# Autodesk Inventor assembly: testframe
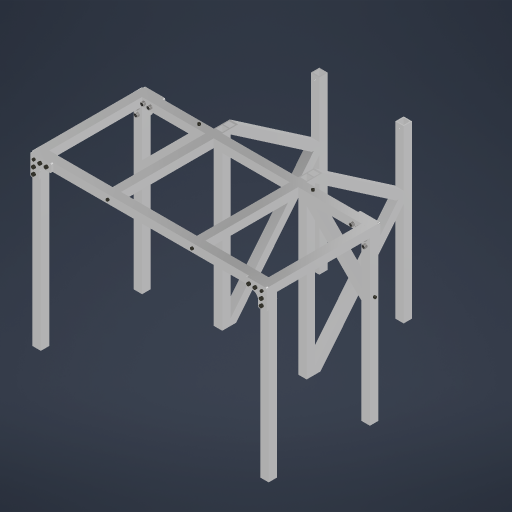
[picture p0: Inventor's stored thumbnail of the model, 512x512]
Saved by Autodesk Inventor 2024.2 (Build 282272000, 272)
## iProperties
Created: 2024-07-23
Part Number: testframe
Document SubType Name: Assembly
Designer: bryan
Mass: 4656.84 g
Surface Area: 9721.76 cm^2
Volume: 1652.17 cm^3
Density: 2.81863 g/cm^3
Author: bryan
## Documents named in this file (24)
- C:\Users\bobsb\OneDrive\Documents\GitHub\1622-2024-Summer-CAD-A-Thon\Structure\STRU_000_StructureAssembly.iam
- C:\Users\bobsb\OneDrive\Documents\GitHub\1622-2024-Summer-CAD-A-Thon\Structure\STRU_001_BilletBlock.ipt
- C:\Users\bobsb\OneDrive\Documents\GitHub\1622-2024-Summer-CAD-A-Thon\Structure\STRU_002_BilletPole_20.56in_Angled.ipt
- C:\Users\bobsb\OneDrive\Documents\GitHub\1622-2024-Summer-CAD-A-Thon\Structure\STRU_003_BilletPole_28in_Angled.ipt
- C:\Users\bobsb\OneDrive\Documents\GitHub\1622-2024-Summer-CAD-A-Thon\Structure\STRU_004_DoubleBillet_90_2.25in.ipt
- C:\Users\bobsb\OneDrive\Documents\GitHub\1622-2024-Summer-CAD-A-Thon\Structure\STRU_007_BilletPole_11in.ipt
- C:\Users\bobsb\OneDrive\Documents\GitHub\1622-2024-Summer-CAD-A-Thon\Structure\STRU_003_BilletPole_28in_Angled_Unique.ipt
- C:\Users\bobsb\OneDrive\Documents\GitHub\1622-2024-Summer-CAD-A-Thon\COTS Library\Fasteners\Bolts\Socket-Head\10-32\COTS_90044A120_Black-Oxide Alloy Steel Socket Head Screw.ipt
- C:\Users\bobsb\OneDrive\Documents\GitHub\1622-2024-Summer-CAD-A-Thon\COTS Library\Fasteners\Bolts\Socket-Head\0.25-20\COTS_90044A123_Black-Oxide Alloy Steel Socket Head Screw.ipt
- C:\Users\bobsb\OneDrive\Documents\GitHub\1622-2024-Summer-CAD-A-Thon\COTS Library\Fasteners\Nuts\COTS_95615A120_Medium-Strength Steel Nylon-Insert Locknut.ipt
- C:\Users\bobsb\OneDrive\Documents\GitHub\1622-2024-Summer-CAD-A-Thon\Structure\STRU_009_FrameBracket_90.ipt
- C:\Users\bobsb\OneDrive\Documents\GitHub\1622-2024-Summer-CAD-A-Thon\Structure\STRU_006_BilletPole_SwerveOffset.ipt
- C:\Users\bobsb\OneDrive\Documents\GitHub\1622-2024-Summer-CAD-A-Thon\Structure\STRU_010_BilletCrossbar_Angled.ipt
- C:\Users\bobsb\OneDrive\Documents\GitHub\1622-2024-Summer-CAD-A-Thon\Structure\STRU_011_BilletWedge.ipt
- C:\Users\bobsb\OneDrive\Documents\GitHub\1622-2024-Summer-CAD-A-Thon\COTS Library\Fasteners\Bolts\Socket-Head\10-32\COTS_90044A119_Black-Oxide Alloy Steel Socket Head Screw.ipt
- C:\Users\bobsb\OneDrive\Documents\GitHub\1622-2024-Summer-CAD-A-Thon\Structure\STRU_012_BilletPoleMiddle.ipt
- C:\Users\bobsb\OneDrive\Documents\GitHub\1622-2024-Summer-CAD-A-Thon\Structure\STRU_013_BilletCrossbar2_Angled.ipt
- C:\Users\bobsb\OneDrive\Documents\GitHub\1622-2024-Summer-CAD-A-Thon\Structure\STRU_014_BilletCrossbar3_Angled.ipt
- C:\Users\bobsb\OneDrive\Documents\GitHub\1622-2024-Summer-CAD-A-Thon\Structure\STRU_000_StructureAssembly\AIP\FEA\err5tqx4w.fins
- C:\Users\bobsb\OneDrive\Documents\GitHub\1622-2024-Summer-CAD-A-Thon\Structure\STRU_000_StructureAssembly\AIP\FEA\err5tqx4w.fsat
- C:\Users\bobsb\OneDrive\Documents\GitHub\1622-2024-Summer-CAD-A-Thon\Structure\STRU_000_StructureAssembly\AIP\FEA\err5tqx4w.ftes
- C:\Users\bobsb\OneDrive\Documents\GitHub\1622-2024-Summer-CAD-A-Thon\Structure\STRU_000_StructureAssembly\AIP\FEA\err5tqx5s.fwiz
- C:\Users\bobsb\OneDrive\Documents\GitHub\1622-2024-Summer-CAD-A-Thon\Structure\STRU_000_StructureAssembly\AIP\FEA\err5tqxb4.fmsh
- C:\Users\bobsb\OneDrive\Documents\GitHub\1622-2024-Summer-CAD-A-Thon\Structure\STRU_000_StructureAssembly\AIP\FEA\err5tqxb5.fres
## Components (90 placed, 17 different names)
1. STRU_001_BilletBlock:2 — Mate:16, Mate:17, Flush:2
2. STRU_002_BilletPole_20.56in_Angled:1 — Mate:1, Mate:4, Mate:5, Mate:41, Mate:53, Mate:54, Flush:10, Mate:91, Mate:92, Mate:127, Mate:147, Mate:148, Mate:199, Mate:209, Mate:211, Mate:212, Mate:213
3. STRU_004_DoubleBillet_90_2.25in:1 — Mate:1, Mate:4, Mate:5, Mate:34, Mate:56, Mate:58, Mate:125, Mate:126
4. STRU_002_BilletPole_20.56in_Angled:2 — Mate:13, Mate:14, Mate:15, Mate:16, Mate:17, Flush:2, Mate:40, Mate:85, Mate:86, Mate:123, Mate:124, Mate:145, Mate:146, Mate:197, Mate:200, Mate:201, Mate:218, Mate:219
5. STRU_004_DoubleBillet_90_2.25in:2 — Mate:13, Mate:14, Mate:15, Mate:36, Mate:57, Mate:100, Mate:121, Mate:122
6. STRU_001_BilletBlock:3 — Mate:185, Mate:186, Flush:26
7. STRU_001_BilletBlock:4 — Mate:180, Mate:181, Flush:25
8. STRU_003_BilletPole_28in_Angled:2 — Mate:47, Flush:8, Flush:9, Mate:55, Mate:74, Mate:79, Mate:80, Mate:87, Mate:88, Mate:97, Mate:118, Mate:130, Mate:140, Mate:153, Mate:154, Mate:155, Mate:156, Mate:157, Mate:158, Mate:161, Mate:163, Mate:168, Mate:173, Flush:24, Mate:176, Mate:178, Mate:182
9. STRU_004_DoubleBillet_90_2.25in:3 — Mate:35, Mate:128, Mate:129, Mate:184
10. STRU_004_DoubleBillet_90_2.25in:4 — Mate:37, Mate:119, Mate:120, Mate:179
11. STRU_001_BilletBlock:5 — Mate:34, Mate:41, Mate:50, Mate:51
12. STRU_001_BilletBlock:6 — Mate:35, Mate:48, Mate:49
13. STRU_001_BilletBlock:7 — Mate:37, Mate:45, Mate:46
14. STRU_001_BilletBlock:8 — Mate:36, Mate:40, Mate:42, Mate:43
15. STRU_007_BilletPole_11in:1 — Mate:48, Mate:49, Flush:9, Mate:50, Mate:51, Mate:55, Mate:59
16. STRU_007_BilletPole_11in:2 — Mate:42, Mate:43, Mate:45, Mate:46, Mate:47, Flush:8, Mate:124
17. STRU_001_BilletBlock:9 — Mate:53, Mate:54, Flush:10
18. STRU_003_BilletPole_28in_Angled_Unique:1 — Mate:56, Mate:57, Mate:58, Mate:59, Mate:83, Mate:84, Mate:93, Mate:94, Mate:98, Mate:149, Mate:150, Mate:151, Mate:152, Mate:159, Mate:160, Mate:164, Mate:165, Mate:196, Mate:198, Flush:27, Mate:203, Mate:205, Mate:206, Mate:208, Mate:214, Mate:215, Mate:216, Mate:217, Mate:220, Flush:28, Mate:221, Mate:222, Flush:29, Mate:223, Flush:35, Mate:232
19. STRU_001_BilletBlock:10 — Mate:74, Mate:157, Mate:172
20. COTS_90044A120_Black-Oxide Alloy Steel Socket Head Screw:1 — Mate:142, Mate:193
21. COTS_90044A123_Black-Oxide Alloy Steel Socket Head Screw:2 — Mate:80, Mate:102, Mate:141, Flush:21
22. COTS_90044A123_Black-Oxide Alloy Steel Socket Head Screw:3 — Mate:103, Flush:22, Flush:23, Mate:191
23. COTS_90044A123_Black-Oxide Alloy Steel Socket Head Screw:4 — Mate:79, Mate:101, Flush:21, Flush:22
24. COTS_90044A123_Black-Oxide Alloy Steel Socket Head Screw:5 — Mate:104, Flush:23, Mate:192
25. COTS_90044A123_Black-Oxide Alloy Steel Socket Head Screw:6 — Mate:84, Mate:108, Flush:12
26. COTS_90044A123_Black-Oxide Alloy Steel Socket Head Screw:7 — Mate:85, Mate:106, Mate:134, Flush:12, Flush:13, Flush:14
27. COTS_90044A123_Black-Oxide Alloy Steel Socket Head Screw:8 — Mate:83, Mate:107, Flush:13
28. COTS_90044A123_Black-Oxide Alloy Steel Socket Head Screw:9 — Mate:86, Mate:105, Flush:14
29. COTS_90044A123_Black-Oxide Alloy Steel Socket Head Screw:10 — Mate:112, Flush:18, Mate:188
30. COTS_90044A123_Black-Oxide Alloy Steel Socket Head Screw:11 — Mate:111, Mate:139, Flush:18, Flush:19, Flush:20, Mate:187
31. COTS_90044A123_Black-Oxide Alloy Steel Socket Head Screw:12 — Mate:88, Mate:110, Flush:20
32. COTS_90044A123_Black-Oxide Alloy Steel Socket Head Screw:13 — Mate:87, Mate:109, Flush:19
33. COTS_90044A123_Black-Oxide Alloy Steel Socket Head Screw:14 — Mate:93, Mate:115, Flush:16
34. COTS_90044A123_Black-Oxide Alloy Steel Socket Head Screw:15 — Mate:92, Mate:114, Flush:17
35. COTS_90044A123_Black-Oxide Alloy Steel Socket Head Screw:16 — Mate:91, Mate:113, Mate:136, Flush:15, Flush:17
36. COTS_90044A123_Black-Oxide Alloy Steel Socket Head Screw:17 — Mate:94, Mate:116, Flush:15, Flush:16
37. COTS_90044A120_Black-Oxide Alloy Steel Socket Head Screw:3 — Mate:140, Mate:158
38. COTS_90044A120_Black-Oxide Alloy Steel Socket Head Screw:5 — Mate:97, Mate:138
39. COTS_90044A120_Black-Oxide Alloy Steel Socket Head Screw:6 — Mate:100, Mate:135
40. COTS_90044A120_Black-Oxide Alloy Steel Socket Head Screw:7 — Mate:98, Mate:137
41. COTS_95615A120_Medium-Strength Steel Nylon-Insert Locknut:1 — Mate:102, Mate:154
42. COTS_95615A120_Medium-Strength Steel Nylon-Insert Locknut:2 — Mate:101, Mate:153
43. COTS_95615A120_Medium-Strength Steel Nylon-Insert Locknut:3 — Mate:103, Mate:194
44. COTS_95615A120_Medium-Strength Steel Nylon-Insert Locknut:4 — Mate:104, Mate:195
45. COTS_95615A120_Medium-Strength Steel Nylon-Insert Locknut:5 — Mate:107, Mate:152
46. COTS_95615A120_Medium-Strength Steel Nylon-Insert Locknut:6 — Mate:108, Mate:151
47. COTS_95615A120_Medium-Strength Steel Nylon-Insert Locknut:7 — Mate:105, Mate:145
48. COTS_95615A120_Medium-Strength Steel Nylon-Insert Locknut:8 — Mate:106, Mate:146
49. COTS_95615A120_Medium-Strength Steel Nylon-Insert Locknut:9 — Mate:109, Mate:155
50. COTS_95615A120_Medium-Strength Steel Nylon-Insert Locknut:10 — Mate:110, Mate:156
51. COTS_95615A120_Medium-Strength Steel Nylon-Insert Locknut:11 — Mate:111, Mate:189
52. COTS_95615A120_Medium-Strength Steel Nylon-Insert Locknut:12 — Mate:112, Mate:190
53. COTS_95615A120_Medium-Strength Steel Nylon-Insert Locknut:13 — Mate:114, Mate:147
54. COTS_95615A120_Medium-Strength Steel Nylon-Insert Locknut:14 — Mate:113, Mate:148
55. COTS_95615A120_Medium-Strength Steel Nylon-Insert Locknut:15 — Mate:115, Mate:149
56. COTS_95615A120_Medium-Strength Steel Nylon-Insert Locknut:16 — Mate:116, Mate:150
57. STRU_009_FrameBracket_90:1 — Mate:118, Mate:119, Mate:120, Mate:141, Mate:142, Mate:177, Mate:191, Mate:192, Mate:193
58. STRU_009_FrameBracket_90:2 — Mate:125, Mate:126, Mate:127, Mate:136, Mate:137
59. STRU_009_FrameBracket_90:3 — Mate:121, Mate:122, Mate:123, Mate:134, Mate:135
60. STRU_009_FrameBracket_90:4 — Mate:128, Mate:129, Mate:130, Mate:138, Mate:139, Mate:183, Mate:187, Mate:188
61. STRU_001_BilletBlock:11 — Mate:159, Mate:165, Mate:171
62. STRU_001_BilletBlock:12 — Mate:160, Mate:164, Mate:174
63. STRU_001_BilletBlock:13 — Mate:161, Mate:162, Mate:163, Mate:175
64. COTS_90044A120_Black-Oxide Alloy Steel Socket Head Screw:10 — Mate:162, Mate:168
65. STRU_007_BilletPole_11in:3 — Mate:171, Mate:172, Mate:173, Flush:27
66. STRU_007_BilletPole_11in:4 — Mate:174, Mate:175, Flush:24, Mate:176
67. STRU_006_BilletPole_SwerveOffset:1 — Mate:177, Mate:178, Mate:179, Mate:180, Mate:181, Flush:25, Mate:194, Mate:195
68. STRU_006_BilletPole_SwerveOffset:2 — Mate:182, Mate:183, Mate:184, Mate:185, Mate:186, Flush:26, Mate:189, Mate:190
69. STRU_010_BilletCrossbar_Angled:1 — Mate:196, Mate:197, Mate:202, Mate:204
70. STRU_010_BilletCrossbar_Angled:2 — Mate:198, Mate:199, Mate:207, Mate:210
71. STRU_011_BilletWedge:1 — Mate:200, Mate:201, Mate:202
72. STRU_011_BilletWedge:3 — Mate:203, Mate:204, Mate:205
73. STRU_011_BilletWedge:4 — Mate:206, Mate:207, Mate:208
74. STRU_011_BilletWedge:5 — Mate:209, Mate:210, Mate:211
75. COTS_90044A119_Black-Oxide Alloy Steel Socket Head Screw:1 — Mate:212, Mate:213
76. COTS_90044A119_Black-Oxide Alloy Steel Socket Head Screw:2 — Mate:214, Mate:215
77. COTS_90044A119_Black-Oxide Alloy Steel Socket Head Screw:3 — Mate:216, Mate:217
78. COTS_90044A119_Black-Oxide Alloy Steel Socket Head Screw:4 — Mate:218, Mate:219
79. STRU_012_BilletPoleMiddle:1 — Mate:220, Flush:28, Mate:221, Mate:228, Mate:229, Flush:30, Flush:34, Flush:43
80. STRU_012_BilletPoleMiddle:2 — Mate:222, Flush:29, Mate:223, Mate:230, Mate:231, Flush:31, Flush:32, Flush:39, Mate:233, Mate:234
81. STRU_001_BilletBlock:14 — Mate:228, Mate:229, Flush:30
82. STRU_001_BilletBlock:15 — Mate:230, Mate:231, Flush:31
83. STRU_012_BilletPoleMiddle:3 — Flush:33, Flush:34, Flush:36, Flush:37, Mate:239, Flush:42, Mate:243, Flush:45, Mate:244, Mate:245, Flush:46
84. STRU_012_BilletPoleMiddle:4 — Flush:32, Flush:33, Flush:35, Flush:36, Mate:232, Flush:37, Mate:241, Flush:44, Mate:246, Mate:247, Flush:47
85. STRU_013_BilletCrossbar2_Angled:1 — Flush:39, Mate:233, Mate:234, Mate:240
86. STRU_013_BilletCrossbar2_Angled:3 — Mate:239, Flush:42, Flush:43, Mate:242
87. STRU_014_BilletCrossbar3_Angled:1 — Mate:240, Mate:241, Flush:44
88. STRU_014_BilletCrossbar3_Angled:2 — Mate:242, Mate:243, Flush:45
89. STRU_001_BilletBlock:16 — Mate:244, Mate:245, Flush:46
90. STRU_001_BilletBlock:17 — Mate:246, Mate:247, Flush:47
## Relationships (218: Mate 181, Flush 37)
- Mate:1: STRU_002_BilletPole_20.56in_Angled:1 ↔ STRU_004_DoubleBillet_90_2.25in:1
- Mate:4: STRU_002_BilletPole_20.56in_Angled:1 ↔ STRU_004_DoubleBillet_90_2.25in:1
- Mate:5: STRU_002_BilletPole_20.56in_Angled:1 ↔ STRU_004_DoubleBillet_90_2.25in:1
- Mate:13: STRU_002_BilletPole_20.56in_Angled:2 ↔ STRU_004_DoubleBillet_90_2.25in:2
- Mate:14: STRU_002_BilletPole_20.56in_Angled:2 ↔ STRU_004_DoubleBillet_90_2.25in:2
- Mate:15: STRU_002_BilletPole_20.56in_Angled:2 ↔ STRU_004_DoubleBillet_90_2.25in:2
- Mate:16: STRU_001_BilletBlock:2 ↔ STRU_002_BilletPole_20.56in_Angled:2
- Mate:17: STRU_001_BilletBlock:2 ↔ STRU_002_BilletPole_20.56in_Angled:2
- Flush:2: STRU_001_BilletBlock:2 ↔ STRU_002_BilletPole_20.56in_Angled:2
- [Mate]: STRU_003_BilletPole_28in_Angled:2 ↔ STRU_004_DoubleBillet_90_2.25in:3
- [Mate]: STRU_003_BilletPole_28in_Angled:2 ↔ STRU_004_DoubleBillet_90_2.25in:3
- [Mate]: STRU_003_BilletPole_28in_Angled:2 ↔ STRU_004_DoubleBillet_90_2.25in:3
- [Mate]: STRU_003_BilletPole_28in_Angled:2 ↔ STRU_004_DoubleBillet_90_2.25in:4
- [Mate]: STRU_003_BilletPole_28in_Angled:2 ↔ STRU_004_DoubleBillet_90_2.25in:4
- [Mate]: STRU_003_BilletPole_28in_Angled:2 ↔ STRU_004_DoubleBillet_90_2.25in:4
- Mate:34: STRU_004_DoubleBillet_90_2.25in:1 ↔ STRU_001_BilletBlock:5
- Mate:35: STRU_004_DoubleBillet_90_2.25in:3 ↔ STRU_001_BilletBlock:6
- Mate:36: STRU_004_DoubleBillet_90_2.25in:2 ↔ STRU_001_BilletBlock:8
- Mate:37: STRU_004_DoubleBillet_90_2.25in:4 ↔ STRU_001_BilletBlock:7
- Mate:40: STRU_002_BilletPole_20.56in_Angled:2 ↔ STRU_001_BilletBlock:8
- Mate:41: STRU_002_BilletPole_20.56in_Angled:1 ↔ STRU_001_BilletBlock:5
- Mate:42: STRU_001_BilletBlock:8 ↔ STRU_007_BilletPole_11in:2
- Mate:43: STRU_001_BilletBlock:8 ↔ STRU_007_BilletPole_11in:2
- Mate:45: STRU_001_BilletBlock:7 ↔ STRU_007_BilletPole_11in:2
- Mate:46: STRU_001_BilletBlock:7 ↔ STRU_007_BilletPole_11in:2
- Mate:47: STRU_003_BilletPole_28in_Angled:2 ↔ STRU_007_BilletPole_11in:2
- Flush:8: STRU_003_BilletPole_28in_Angled:2 ↔ STRU_007_BilletPole_11in:2
- Mate:48: STRU_001_BilletBlock:6 ↔ STRU_007_BilletPole_11in:1
- Mate:49: STRU_001_BilletBlock:6 ↔ STRU_007_BilletPole_11in:1
- Flush:9: STRU_003_BilletPole_28in_Angled:2 ↔ STRU_007_BilletPole_11in:1
- Mate:50: STRU_001_BilletBlock:5 ↔ STRU_007_BilletPole_11in:1
- Mate:51: STRU_001_BilletBlock:5 ↔ STRU_007_BilletPole_11in:1
- Mate:53: STRU_002_BilletPole_20.56in_Angled:1 ↔ STRU_001_BilletBlock:9
- Mate:54: STRU_002_BilletPole_20.56in_Angled:1 ↔ STRU_001_BilletBlock:9
- Flush:10: STRU_002_BilletPole_20.56in_Angled:1 ↔ STRU_001_BilletBlock:9
- Mate:55: STRU_003_BilletPole_28in_Angled:2 ↔ STRU_007_BilletPole_11in:1
- Mate:56: STRU_004_DoubleBillet_90_2.25in:1 ↔ STRU_003_BilletPole_28in_Angled_Unique:1
- Mate:57: STRU_004_DoubleBillet_90_2.25in:2 ↔ STRU_003_BilletPole_28in_Angled_Unique:1
- Mate:58: STRU_004_DoubleBillet_90_2.25in:1 ↔ STRU_003_BilletPole_28in_Angled_Unique:1
- Mate:59: STRU_007_BilletPole_11in:1 ↔ STRU_003_BilletPole_28in_Angled_Unique:1
- Mate:74: STRU_003_BilletPole_28in_Angled:2 ↔ STRU_001_BilletBlock:10
- Mate:79: STRU_003_BilletPole_28in_Angled:2 ↔ COTS_90044A123_Black-Oxide Alloy Steel Socket Head Screw:4
- Mate:80: STRU_003_BilletPole_28in_Angled:2 ↔ COTS_90044A123_Black-Oxide Alloy Steel Socket Head Screw:2
- Mate:83: STRU_003_BilletPole_28in_Angled_Unique:1 ↔ COTS_90044A123_Black-Oxide Alloy Steel Socket Head Screw:8
- Mate:84: STRU_003_BilletPole_28in_Angled_Unique:1 ↔ COTS_90044A123_Black-Oxide Alloy Steel Socket Head Screw:6
- Mate:85: STRU_002_BilletPole_20.56in_Angled:2 ↔ COTS_90044A123_Black-Oxide Alloy Steel Socket Head Screw:7
- Mate:86: STRU_002_BilletPole_20.56in_Angled:2 ↔ COTS_90044A123_Black-Oxide Alloy Steel Socket Head Screw:9
- Mate:87: STRU_003_BilletPole_28in_Angled:2 ↔ COTS_90044A123_Black-Oxide Alloy Steel Socket Head Screw:13
- Mate:88: STRU_003_BilletPole_28in_Angled:2 ↔ COTS_90044A123_Black-Oxide Alloy Steel Socket Head Screw:12
- Mate:91: STRU_002_BilletPole_20.56in_Angled:1 ↔ COTS_90044A123_Black-Oxide Alloy Steel Socket Head Screw:16
- Mate:92: STRU_002_BilletPole_20.56in_Angled:1 ↔ COTS_90044A123_Black-Oxide Alloy Steel Socket Head Screw:15
- Mate:93: STRU_003_BilletPole_28in_Angled_Unique:1 ↔ COTS_90044A123_Black-Oxide Alloy Steel Socket Head Screw:14
- Mate:94: STRU_003_BilletPole_28in_Angled_Unique:1 ↔ COTS_90044A123_Black-Oxide Alloy Steel Socket Head Screw:17
- Mate:97: STRU_003_BilletPole_28in_Angled:2 ↔ COTS_90044A120_Black-Oxide Alloy Steel Socket Head Screw:5
- Mate:98: STRU_003_BilletPole_28in_Angled_Unique:1 ↔ COTS_90044A120_Black-Oxide Alloy Steel Socket Head Screw:7
- Mate:100: STRU_004_DoubleBillet_90_2.25in:2 ↔ COTS_90044A120_Black-Oxide Alloy Steel Socket Head Screw:6
- Mate:101: COTS_90044A123_Black-Oxide Alloy Steel Socket Head Screw:4 ↔ COTS_95615A120_Medium-Strength Steel Nylon-Insert Locknut:2
- Mate:102: COTS_90044A123_Black-Oxide Alloy Steel Socket Head Screw:2 ↔ COTS_95615A120_Medium-Strength Steel Nylon-Insert Locknut:1
- Mate:103: COTS_90044A123_Black-Oxide Alloy Steel Socket Head Screw:3 ↔ COTS_95615A120_Medium-Strength Steel Nylon-Insert Locknut:3
- Mate:104: COTS_90044A123_Black-Oxide Alloy Steel Socket Head Screw:5 ↔ COTS_95615A120_Medium-Strength Steel Nylon-Insert Locknut:4
- Mate:105: COTS_90044A123_Black-Oxide Alloy Steel Socket Head Screw:9 ↔ COTS_95615A120_Medium-Strength Steel Nylon-Insert Locknut:7
- Mate:106: COTS_90044A123_Black-Oxide Alloy Steel Socket Head Screw:7 ↔ COTS_95615A120_Medium-Strength Steel Nylon-Insert Locknut:8
- Mate:107: COTS_90044A123_Black-Oxide Alloy Steel Socket Head Screw:8 ↔ COTS_95615A120_Medium-Strength Steel Nylon-Insert Locknut:5
- Mate:108: COTS_90044A123_Black-Oxide Alloy Steel Socket Head Screw:6 ↔ COTS_95615A120_Medium-Strength Steel Nylon-Insert Locknut:6
- Mate:109: COTS_90044A123_Black-Oxide Alloy Steel Socket Head Screw:13 ↔ COTS_95615A120_Medium-Strength Steel Nylon-Insert Locknut:9
- Mate:110: COTS_90044A123_Black-Oxide Alloy Steel Socket Head Screw:12 ↔ COTS_95615A120_Medium-Strength Steel Nylon-Insert Locknut:10
- Mate:111: COTS_90044A123_Black-Oxide Alloy Steel Socket Head Screw:11 ↔ COTS_95615A120_Medium-Strength Steel Nylon-Insert Locknut:11
- Mate:112: COTS_90044A123_Black-Oxide Alloy Steel Socket Head Screw:10 ↔ COTS_95615A120_Medium-Strength Steel Nylon-Insert Locknut:12
- Mate:113: COTS_90044A123_Black-Oxide Alloy Steel Socket Head Screw:16 ↔ COTS_95615A120_Medium-Strength Steel Nylon-Insert Locknut:14
- Mate:114: COTS_90044A123_Black-Oxide Alloy Steel Socket Head Screw:15 ↔ COTS_95615A120_Medium-Strength Steel Nylon-Insert Locknut:13
- Mate:115: COTS_90044A123_Black-Oxide Alloy Steel Socket Head Screw:14 ↔ COTS_95615A120_Medium-Strength Steel Nylon-Insert Locknut:15
- Mate:116: COTS_90044A123_Black-Oxide Alloy Steel Socket Head Screw:17 ↔ COTS_95615A120_Medium-Strength Steel Nylon-Insert Locknut:16
- Mate:118: STRU_003_BilletPole_28in_Angled:2 ↔ STRU_009_FrameBracket_90:1
- Mate:119: STRU_004_DoubleBillet_90_2.25in:4 ↔ STRU_009_FrameBracket_90:1
- Mate:120: STRU_004_DoubleBillet_90_2.25in:4 ↔ STRU_009_FrameBracket_90:1
- Mate:121: STRU_004_DoubleBillet_90_2.25in:2 ↔ STRU_009_FrameBracket_90:3
- Mate:122: STRU_004_DoubleBillet_90_2.25in:2 ↔ STRU_009_FrameBracket_90:3
- Mate:123: STRU_002_BilletPole_20.56in_Angled:2 ↔ STRU_009_FrameBracket_90:3
- Mate:124: STRU_002_BilletPole_20.56in_Angled:2 ↔ STRU_007_BilletPole_11in:2
- Mate:125: STRU_004_DoubleBillet_90_2.25in:1 ↔ STRU_009_FrameBracket_90:2
- Mate:126: STRU_004_DoubleBillet_90_2.25in:1 ↔ STRU_009_FrameBracket_90:2
- Mate:127: STRU_002_BilletPole_20.56in_Angled:1 ↔ STRU_009_FrameBracket_90:2
- Mate:128: STRU_004_DoubleBillet_90_2.25in:3 ↔ STRU_009_FrameBracket_90:4
- Mate:129: STRU_004_DoubleBillet_90_2.25in:3 ↔ STRU_009_FrameBracket_90:4
- Mate:130: STRU_003_BilletPole_28in_Angled:2 ↔ STRU_009_FrameBracket_90:4
- Mate:134: COTS_90044A123_Black-Oxide Alloy Steel Socket Head Screw:7 ↔ STRU_009_FrameBracket_90:3
- Flush:12: COTS_90044A123_Black-Oxide Alloy Steel Socket Head Screw:6 ↔ COTS_90044A123_Black-Oxide Alloy Steel Socket Head Screw:7
- Mate:135: COTS_90044A120_Black-Oxide Alloy Steel Socket Head Screw:6 ↔ STRU_009_FrameBracket_90:3
- Flush:13: COTS_90044A123_Black-Oxide Alloy Steel Socket Head Screw:7 ↔ COTS_90044A123_Black-Oxide Alloy Steel Socket Head Screw:8
- Flush:14: COTS_90044A123_Black-Oxide Alloy Steel Socket Head Screw:7 ↔ COTS_90044A123_Black-Oxide Alloy Steel Socket Head Screw:9
- Mate:136: COTS_90044A123_Black-Oxide Alloy Steel Socket Head Screw:16 ↔ STRU_009_FrameBracket_90:2
- Mate:137: COTS_90044A120_Black-Oxide Alloy Steel Socket Head Screw:7 ↔ STRU_009_FrameBracket_90:2
- Flush:15: COTS_90044A123_Black-Oxide Alloy Steel Socket Head Screw:16 ↔ COTS_90044A123_Black-Oxide Alloy Steel Socket Head Screw:17
- Flush:16: COTS_90044A123_Black-Oxide Alloy Steel Socket Head Screw:14 ↔ COTS_90044A123_Black-Oxide Alloy Steel Socket Head Screw:17
- Flush:17: COTS_90044A123_Black-Oxide Alloy Steel Socket Head Screw:15 ↔ COTS_90044A123_Black-Oxide Alloy Steel Socket Head Screw:16
- Mate:138: COTS_90044A120_Black-Oxide Alloy Steel Socket Head Screw:5 ↔ STRU_009_FrameBracket_90:4
- Mate:139: COTS_90044A123_Black-Oxide Alloy Steel Socket Head Screw:11 ↔ STRU_009_FrameBracket_90:4
- Flush:18: COTS_90044A123_Black-Oxide Alloy Steel Socket Head Screw:10 ↔ COTS_90044A123_Black-Oxide Alloy Steel Socket Head Screw:11
- Flush:19: COTS_90044A123_Black-Oxide Alloy Steel Socket Head Screw:11 ↔ COTS_90044A123_Black-Oxide Alloy Steel Socket Head Screw:13
- Flush:20: COTS_90044A123_Black-Oxide Alloy Steel Socket Head Screw:11 ↔ COTS_90044A123_Black-Oxide Alloy Steel Socket Head Screw:12
- Mate:140: STRU_003_BilletPole_28in_Angled:2 ↔ COTS_90044A120_Black-Oxide Alloy Steel Socket Head Screw:3
- Mate:141: COTS_90044A123_Black-Oxide Alloy Steel Socket Head Screw:2 ↔ STRU_009_FrameBracket_90:1
- Mate:142: COTS_90044A120_Black-Oxide Alloy Steel Socket Head Screw:1 ↔ STRU_009_FrameBracket_90:1
- Flush:21: COTS_90044A123_Black-Oxide Alloy Steel Socket Head Screw:2 ↔ COTS_90044A123_Black-Oxide Alloy Steel Socket Head Screw:4
- Flush:22: COTS_90044A123_Black-Oxide Alloy Steel Socket Head Screw:3 ↔ COTS_90044A123_Black-Oxide Alloy Steel Socket Head Screw:4
- Flush:23: COTS_90044A123_Black-Oxide Alloy Steel Socket Head Screw:3 ↔ COTS_90044A123_Black-Oxide Alloy Steel Socket Head Screw:5
- Mate:145: STRU_002_BilletPole_20.56in_Angled:2 ↔ COTS_95615A120_Medium-Strength Steel Nylon-Insert Locknut:7
- Mate:146: STRU_002_BilletPole_20.56in_Angled:2 ↔ COTS_95615A120_Medium-Strength Steel Nylon-Insert Locknut:8
- Mate:147: STRU_002_BilletPole_20.56in_Angled:1 ↔ COTS_95615A120_Medium-Strength Steel Nylon-Insert Locknut:13
- Mate:148: STRU_002_BilletPole_20.56in_Angled:1 ↔ COTS_95615A120_Medium-Strength Steel Nylon-Insert Locknut:14
- Mate:149: STRU_003_BilletPole_28in_Angled_Unique:1 ↔ COTS_95615A120_Medium-Strength Steel Nylon-Insert Locknut:15
- Mate:150: STRU_003_BilletPole_28in_Angled_Unique:1 ↔ COTS_95615A120_Medium-Strength Steel Nylon-Insert Locknut:16
- Mate:151: STRU_003_BilletPole_28in_Angled_Unique:1 ↔ COTS_95615A120_Medium-Strength Steel Nylon-Insert Locknut:6
- Mate:152: STRU_003_BilletPole_28in_Angled_Unique:1 ↔ COTS_95615A120_Medium-Strength Steel Nylon-Insert Locknut:5
- Mate:153: STRU_003_BilletPole_28in_Angled:2 ↔ COTS_95615A120_Medium-Strength Steel Nylon-Insert Locknut:2
- Mate:154: STRU_003_BilletPole_28in_Angled:2 ↔ COTS_95615A120_Medium-Strength Steel Nylon-Insert Locknut:1
- Mate:155: STRU_003_BilletPole_28in_Angled:2 ↔ COTS_95615A120_Medium-Strength Steel Nylon-Insert Locknut:9
- Mate:156: STRU_003_BilletPole_28in_Angled:2 ↔ COTS_95615A120_Medium-Strength Steel Nylon-Insert Locknut:10
- Mate:157: STRU_003_BilletPole_28in_Angled:2 ↔ STRU_001_BilletBlock:10
- Mate:158: STRU_003_BilletPole_28in_Angled:2 ↔ COTS_90044A120_Black-Oxide Alloy Steel Socket Head Screw:3
- Mate:159: STRU_003_BilletPole_28in_Angled_Unique:1 ↔ STRU_001_BilletBlock:11
- Mate:160: STRU_003_BilletPole_28in_Angled_Unique:1 ↔ STRU_001_BilletBlock:12
- Mate:161: STRU_003_BilletPole_28in_Angled:2 ↔ STRU_001_BilletBlock:13
- Mate:162: STRU_001_BilletBlock:13 ↔ COTS_90044A120_Black-Oxide Alloy Steel Socket Head Screw:10
- Mate:163: STRU_003_BilletPole_28in_Angled:2 ↔ STRU_001_BilletBlock:13
- Mate:164: STRU_003_BilletPole_28in_Angled_Unique:1 ↔ STRU_001_BilletBlock:12
- Mate:165: STRU_003_BilletPole_28in_Angled_Unique:1 ↔ STRU_001_BilletBlock:11
- Mate:168: STRU_003_BilletPole_28in_Angled:2 ↔ COTS_90044A120_Black-Oxide Alloy Steel Socket Head Screw:10
- Mate:171: STRU_001_BilletBlock:11 ↔ STRU_007_BilletPole_11in:3
- Mate:172: STRU_001_BilletBlock:10 ↔ STRU_007_BilletPole_11in:3
- Mate:173: STRU_003_BilletPole_28in_Angled:2 ↔ STRU_007_BilletPole_11in:3
- Mate:174: STRU_001_BilletBlock:12 ↔ STRU_007_BilletPole_11in:4
- Mate:175: STRU_001_BilletBlock:13 ↔ STRU_007_BilletPole_11in:4
- Flush:24: STRU_003_BilletPole_28in_Angled:2 ↔ STRU_007_BilletPole_11in:4
- Mate:176: STRU_003_BilletPole_28in_Angled:2 ↔ STRU_007_BilletPole_11in:4
- Mate:177: STRU_009_FrameBracket_90:1 ↔ STRU_006_BilletPole_SwerveOffset:1
- Mate:178: STRU_003_BilletPole_28in_Angled:2 ↔ STRU_006_BilletPole_SwerveOffset:1
- Mate:179: STRU_004_DoubleBillet_90_2.25in:4 ↔ STRU_006_BilletPole_SwerveOffset:1
- Mate:180: STRU_001_BilletBlock:4 ↔ STRU_006_BilletPole_SwerveOffset:1
- Mate:181: STRU_001_BilletBlock:4 ↔ STRU_006_BilletPole_SwerveOffset:1
- Flush:25: STRU_001_BilletBlock:4 ↔ STRU_006_BilletPole_SwerveOffset:1
- Mate:182: STRU_003_BilletPole_28in_Angled:2 ↔ STRU_006_BilletPole_SwerveOffset:2
- Mate:183: STRU_009_FrameBracket_90:4 ↔ STRU_006_BilletPole_SwerveOffset:2
- Mate:184: STRU_004_DoubleBillet_90_2.25in:3 ↔ STRU_006_BilletPole_SwerveOffset:2
- Mate:185: STRU_001_BilletBlock:3 ↔ STRU_006_BilletPole_SwerveOffset:2
- Mate:186: STRU_001_BilletBlock:3 ↔ STRU_006_BilletPole_SwerveOffset:2
- Flush:26: STRU_001_BilletBlock:3 ↔ STRU_006_BilletPole_SwerveOffset:2
- Mate:187: COTS_90044A123_Black-Oxide Alloy Steel Socket Head Screw:11 ↔ STRU_009_FrameBracket_90:4
- Mate:188: COTS_90044A123_Black-Oxide Alloy Steel Socket Head Screw:10 ↔ STRU_009_FrameBracket_90:4
- Mate:189: COTS_95615A120_Medium-Strength Steel Nylon-Insert Locknut:11 ↔ STRU_006_BilletPole_SwerveOffset:2
- Mate:190: COTS_95615A120_Medium-Strength Steel Nylon-Insert Locknut:12 ↔ STRU_006_BilletPole_SwerveOffset:2
- Mate:191: COTS_90044A123_Black-Oxide Alloy Steel Socket Head Screw:3 ↔ STRU_009_FrameBracket_90:1
- Mate:192: COTS_90044A123_Black-Oxide Alloy Steel Socket Head Screw:5 ↔ STRU_009_FrameBracket_90:1
- Mate:193: COTS_90044A120_Black-Oxide Alloy Steel Socket Head Screw:1 ↔ STRU_009_FrameBracket_90:1
- Mate:194: COTS_95615A120_Medium-Strength Steel Nylon-Insert Locknut:3 ↔ STRU_006_BilletPole_SwerveOffset:1
- Mate:195: COTS_95615A120_Medium-Strength Steel Nylon-Insert Locknut:4 ↔ STRU_006_BilletPole_SwerveOffset:1
- Mate:196: STRU_003_BilletPole_28in_Angled_Unique:1 ↔ STRU_010_BilletCrossbar_Angled:1
- Mate:197: STRU_002_BilletPole_20.56in_Angled:2 ↔ STRU_010_BilletCrossbar_Angled:1
- Mate:198: STRU_003_BilletPole_28in_Angled_Unique:1 ↔ STRU_010_BilletCrossbar_Angled:2
- Mate:199: STRU_002_BilletPole_20.56in_Angled:1 ↔ STRU_010_BilletCrossbar_Angled:2
- Flush:27: STRU_003_BilletPole_28in_Angled_Unique:1 ↔ STRU_007_BilletPole_11in:3
- Mate:200: STRU_002_BilletPole_20.56in_Angled:2 ↔ STRU_011_BilletWedge:1
- Mate:201: STRU_002_BilletPole_20.56in_Angled:2 ↔ STRU_011_BilletWedge:1
- Mate:202: STRU_010_BilletCrossbar_Angled:1 ↔ STRU_011_BilletWedge:1
- Mate:203: STRU_003_BilletPole_28in_Angled_Unique:1 ↔ STRU_011_BilletWedge:3
- Mate:204: STRU_010_BilletCrossbar_Angled:1 ↔ STRU_011_BilletWedge:3
- Mate:205: STRU_003_BilletPole_28in_Angled_Unique:1 ↔ STRU_011_BilletWedge:3
- Mate:206: STRU_003_BilletPole_28in_Angled_Unique:1 ↔ STRU_011_BilletWedge:4
- Mate:207: STRU_010_BilletCrossbar_Angled:2 ↔ STRU_011_BilletWedge:4
- Mate:208: STRU_003_BilletPole_28in_Angled_Unique:1 ↔ STRU_011_BilletWedge:4
- Mate:209: STRU_002_BilletPole_20.56in_Angled:1 ↔ STRU_011_BilletWedge:5
- Mate:210: STRU_010_BilletCrossbar_Angled:2 ↔ STRU_011_BilletWedge:5
- Mate:211: STRU_002_BilletPole_20.56in_Angled:1 ↔ STRU_011_BilletWedge:5
- Mate:212: STRU_002_BilletPole_20.56in_Angled:1 ↔ COTS_90044A119_Black-Oxide Alloy Steel Socket Head Screw:1
- Mate:213: STRU_002_BilletPole_20.56in_Angled:1 ↔ COTS_90044A119_Black-Oxide Alloy Steel Socket Head Screw:1
- Mate:214: STRU_003_BilletPole_28in_Angled_Unique:1 ↔ COTS_90044A119_Black-Oxide Alloy Steel Socket Head Screw:2
- Mate:215: STRU_003_BilletPole_28in_Angled_Unique:1 ↔ COTS_90044A119_Black-Oxide Alloy Steel Socket Head Screw:2
- Mate:216: STRU_003_BilletPole_28in_Angled_Unique:1 ↔ COTS_90044A119_Black-Oxide Alloy Steel Socket Head Screw:3
- Mate:217: STRU_003_BilletPole_28in_Angled_Unique:1 ↔ COTS_90044A119_Black-Oxide Alloy Steel Socket Head Screw:3
- Mate:218: STRU_002_BilletPole_20.56in_Angled:2 ↔ COTS_90044A119_Black-Oxide Alloy Steel Socket Head Screw:4
- Mate:219: STRU_002_BilletPole_20.56in_Angled:2 ↔ COTS_90044A119_Black-Oxide Alloy Steel Socket Head Screw:4
- Mate:220: STRU_003_BilletPole_28in_Angled_Unique:1 ↔ STRU_012_BilletPoleMiddle:1
- Flush:28: STRU_003_BilletPole_28in_Angled_Unique:1 ↔ STRU_012_BilletPoleMiddle:1
- Mate:221: STRU_003_BilletPole_28in_Angled_Unique:1 ↔ STRU_012_BilletPoleMiddle:1
- Mate:222: STRU_003_BilletPole_28in_Angled_Unique:1 ↔ STRU_012_BilletPoleMiddle:2
- Flush:29: STRU_003_BilletPole_28in_Angled_Unique:1 ↔ STRU_012_BilletPoleMiddle:2
- Mate:223: STRU_003_BilletPole_28in_Angled_Unique:1 ↔ STRU_012_BilletPoleMiddle:2
- Mate:228: STRU_012_BilletPoleMiddle:1 ↔ STRU_001_BilletBlock:14
- Mate:229: STRU_012_BilletPoleMiddle:1 ↔ STRU_001_BilletBlock:14
- Flush:30: STRU_012_BilletPoleMiddle:1 ↔ STRU_001_BilletBlock:14
- Mate:230: STRU_012_BilletPoleMiddle:2 ↔ STRU_001_BilletBlock:15
- Mate:231: STRU_012_BilletPoleMiddle:2 ↔ STRU_001_BilletBlock:15
- Flush:31: STRU_012_BilletPoleMiddle:2 ↔ STRU_001_BilletBlock:15
- Flush:32: STRU_012_BilletPoleMiddle:2 ↔ STRU_012_BilletPoleMiddle:4
- Flush:33: STRU_012_BilletPoleMiddle:3 ↔ STRU_012_BilletPoleMiddle:4
- Flush:34: STRU_012_BilletPoleMiddle:1 ↔ STRU_012_BilletPoleMiddle:3
- Flush:35: STRU_003_BilletPole_28in_Angled_Unique:1 ↔ STRU_012_BilletPoleMiddle:4
- Flush:36: STRU_012_BilletPoleMiddle:3 ↔ STRU_012_BilletPoleMiddle:4
- Mate:232 (292.1 mm): STRU_003_BilletPole_28in_Angled_Unique:1 ↔ STRU_012_BilletPoleMiddle:4
- Flush:37: STRU_012_BilletPoleMiddle:3 ↔ STRU_012_BilletPoleMiddle:4
- Flush:39: STRU_012_BilletPoleMiddle:2 ↔ STRU_013_BilletCrossbar2_Angled:1
- Mate:233: STRU_012_BilletPoleMiddle:2 ↔ STRU_013_BilletCrossbar2_Angled:1
- Mate:234: STRU_012_BilletPoleMiddle:2 ↔ STRU_013_BilletCrossbar2_Angled:1
- Mate:239: STRU_012_BilletPoleMiddle:3 ↔ STRU_013_BilletCrossbar2_Angled:3
- Flush:42: STRU_012_BilletPoleMiddle:3 ↔ STRU_013_BilletCrossbar2_Angled:3
- Flush:43: STRU_012_BilletPoleMiddle:1 ↔ STRU_013_BilletCrossbar2_Angled:3
- Mate:240: STRU_013_BilletCrossbar2_Angled:1 ↔ STRU_014_BilletCrossbar3_Angled:1
- Mate:241: STRU_012_BilletPoleMiddle:4 ↔ STRU_014_BilletCrossbar3_Angled:1
- Flush:44: STRU_012_BilletPoleMiddle:4 ↔ STRU_014_BilletCrossbar3_Angled:1
- Mate:242: STRU_013_BilletCrossbar2_Angled:3 ↔ STRU_014_BilletCrossbar3_Angled:2
- Mate:243: STRU_012_BilletPoleMiddle:3 ↔ STRU_014_BilletCrossbar3_Angled:2
- Flush:45: STRU_012_BilletPoleMiddle:3 ↔ STRU_014_BilletCrossbar3_Angled:2
- Mate:244: STRU_012_BilletPoleMiddle:3 ↔ STRU_001_BilletBlock:16
- Mate:245: STRU_012_BilletPoleMiddle:3 ↔ STRU_001_BilletBlock:16
- Flush:46: STRU_012_BilletPoleMiddle:3 ↔ STRU_001_BilletBlock:16
- Mate:246: STRU_012_BilletPoleMiddle:4 ↔ STRU_001_BilletBlock:17
- Mate:247: STRU_012_BilletPoleMiddle:4 ↔ STRU_001_BilletBlock:17
- Flush:47: STRU_012_BilletPoleMiddle:4 ↔ STRU_001_BilletBlock:17
## Named parameters: d22_d7 = 0 mm, d23_d8 = 0 mm, d24_d9 = 0 mm, d25_d10 = 0 mm, d26_d11 = 0 mm, d27_d12 = 0 mm, sa_0 = 4448.22, sa_1 = 4448.22
note: some values were not read from the file. Shown as the stored number, unit unknown: "sa_0", "sa_1".
